# Autodesk Inventor assembly: CE-9.1.2
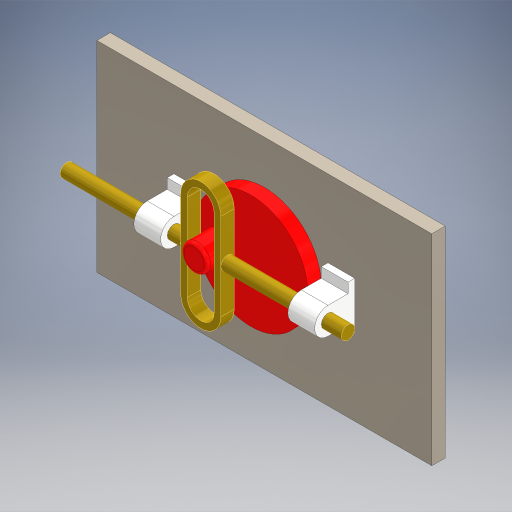
[picture p0: Inventor's stored thumbnail of the model, 512x512]
Saved by Autodesk Inventor 2024 (Build 280153000, 153)
## iProperties
Created: 2024-03-14
Part Number: CE-9.1.2
Document SubType Name: Assembly
Designer: Alex
Author: Alex
## Documents named in this file (4)
- C:\Shared\alex-bartella-schoolwork\4z03\Week 9\CE-9.1.2.iam
- C:\Shared\alex-bartella-schoolwork\4z03\Week 9\STEP\CE-9.1.1 STEP Files\base\base.ipt
- C:\Shared\alex-bartella-schoolwork\4z03\Week 9\STEP\CE-9.1.1 STEP Files\disk\disk.ipt
- C:\Shared\alex-bartella-schoolwork\4z03\Week 9\STEP\CE-9.1.1 STEP Files\slotted_bar\slotted_bar.ipt
## Components (3 placed, 3 different names)
1. base:1 — Mate:1, Flush:1, Flush:2, Flush:3, Mate:2, Mate:3, Angle:1, Angle:2
2. disk:1 — Mate:2, Mate:3, Transitional:1, Angle:2
3. slotted_bar:1 — Mate:1, Angle:1, Transitional:1
## Relationships (9: Mate 3, Flush 3, Angle 2, Transitional 1)
- Mate:1: base:1 ↔ slotted_bar:1
- Flush:1: base:1
- Flush:2: base:1
- Flush:3: base:1
- Mate:2: base:1 ↔ disk:1
- Mate:3: base:1 ↔ disk:1
- Angle:1 (0 deg): base:1 ↔ slotted_bar:1
- Transitional:1: disk:1 ↔ slotted_bar:1
- Angle:2 (900 deg): base:1 ↔ disk:1
